# Autodesk Inventor assembly: 2.75 Traction AS, No Insert_MIR
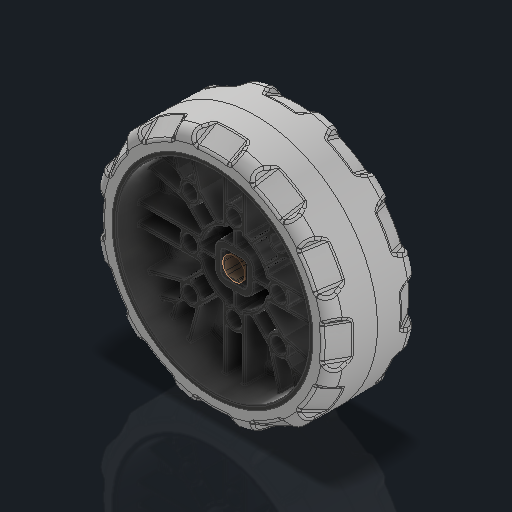
[picture p0: Inventor's stored thumbnail of the model, 512x512]
Saved by Autodesk Inventor 2023.2 (Build 272271030, 271C)
## iProperties
Created: 2022-08-02
Part Number: 2.75 Traction AS, No Insert_MIR
Document SubType Name: Assembly
Designer: Michael
Author: ylu12
## Documents named in this file (2)
- C:\Users\black\OneDrive\Pictures\Documents\VEX CAD\VEX-CAD-Inventor-1.4.0\Motion\Wheels\Traction Wheel\2.75 Traction AS, No Insert_MIR.iam
- C:\Users\black\OneDrive\Pictures\Documents\VEX CAD\VEX-CAD-Inventor-1.4.0\Motion\Wheels\Reference Files\2.75 Traction Antistatic_MIR.ipt
## Components (1 placed, 1 different names)
1. 2.75 Traction Antistatic_MIR:1 — Mate:19, Mate:18, Mate:17
## Relationships (3: Flush 2, Mate 1)
- Mate:19 [Flush]: 2.75 Traction Antistatic_MIR:1
- Mate:18 [Flush]: 2.75 Traction Antistatic_MIR:1
- Mate:17: 2.75 Traction Antistatic_MIR:1
## Named parameters: Thickness = 8.255 mm
